# Autodesk Inventor assembly: 047117-1880 REAR HEAD COVER-ASSY-3
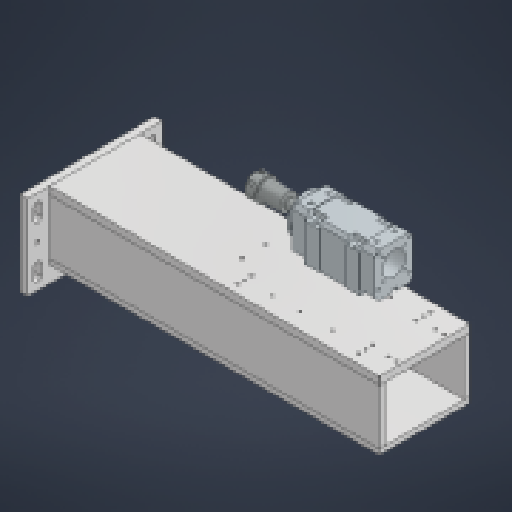
[picture p0: Inventor's stored thumbnail of the model, 512x512]
Saved by Autodesk Inventor 2026.2 (Build 302298000, 298)
## iProperties
Created: 2025-11-25
Part Number: 047117-1880 REAR HEAD COVER-ASSY-3
Document SubType Name: Assembly
Designer: USUARIO
Author: USUARIO
## Documents named in this file (7)
- F:\UNAL\14. SEMESTRE\AUTOMATIZACIÓN DE PROCESOS DE MANUFACTURA\GitHub\Los4Automaticos\CAD\InventorProyecto\Taladro\Taladro\047117-1880 REAR HEAD COVER-ASSY-3.iam
- F:\UNAL\14. SEMESTRE\AUTOMATIZACIÓN DE PROCESOS DE MANUFACTURA\GitHub\Los4Automaticos\CAD\InventorProyecto\Taladro\Taladro\047119-405_0-00-P-10.ipt
- F:\UNAL\14. SEMESTRE\AUTOMATIZACIÓN DE PROCESOS DE MANUFACTURA\GitHub\Los4Automaticos\CAD\InventorProyecto\Taladro\Taladro\047119-405_0-00-P-10_1.ipt
- F:\UNAL\14. SEMESTRE\AUTOMATIZACIÓN DE PROCESOS DE MANUFACTURA\GitHub\Los4Automaticos\CAD\InventorProyecto\Taladro\Taladro\047119-405_0-00-P-10_2.ipt
- F:\UNAL\14. SEMESTRE\AUTOMATIZACIÓN DE PROCESOS DE MANUFACTURA\GitHub\Los4Automaticos\CAD\InventorProyecto\Taladro\Taladro\047119-405_0-00-P-10_3.ipt
- F:\UNAL\14. SEMESTRE\AUTOMATIZACIÓN DE PROCESOS DE MANUFACTURA\GitHub\Los4Automaticos\CAD\InventorProyecto\Taladro\Taladro\047119-405_0-00-P-10_4.ipt
- F:\UNAL\14. SEMESTRE\AUTOMATIZACIÓN DE PROCESOS DE MANUFACTURA\GitHub\Los4Automaticos\CAD\InventorProyecto\Taladro\Taladro\S25-MB-ER20-000-11.iam
## Components (6 placed, 6 different names)
1. 047119-405_0-00-P-10
2. 047119-405_0-00-P-10_1
3. 047119-405_0-00-P-10_2
4. 047119-405_0-00-P-10_3
5. 047119-405_0-00-P-10_4 — Coincidencia:1
6. S25-MB-ER20-000-11 [sub-assembly] — Coincidencia:1
## Relationships (1: Mate 1)
- Coincidencia:1 [Mate]: 047119-405_0-00-P-10_4 ↔ S25-MB-ER20-000-11
